# Autodesk Inventor assembly: Assembly1
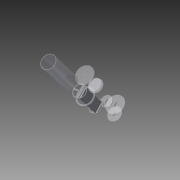
[picture p0: Inventor's stored thumbnail of the model, 180x180]
Saved by Autodesk Inventor 2015 (Build 190159000, 159)
## iProperties
Created: 2015-02-17
Part Number: Assembly1
Document SubType Name: Assembly
Designer: Hanjie
Author: Hanjie
## Documents named in this file (14)
- C:\Users\Qiuyang\Dropbox\VIP\SeaPerch\Dimensions\tube\Assembly1.iam
- C:\Users\Qiuyang\Dropbox\VIP\SeaPerch\Dimensions\tube\seal1.ipt
- C:\Users\Qiuyang\Dropbox\VIP\SeaPerch\Dimensions\tube\seal2.ipt
- C:\Users\Qiuyang\Dropbox\VIP\SeaPerch\Dimensions\tube\seal3.ipt
- C:\Users\Qiuyang\Dropbox\VIP\SeaPerch\Dimensions\tube\tube.ipt
- C:\Users\Qiuyang\Dropbox\VIP\SeaPerch\Dimensions\tube\open1.ipt
- C:\Users\Qiuyang\Dropbox\VIP\SeaPerch\Dimensions\tube\open2.ipt
- C:\Users\Qiuyang\Dropbox\VIP\SeaPerch\Dimensions\tube\open3.ipt
- C:\Users\Qiuyang\Dropbox\VIP\SeaPerch\Dimensions\tube\open4.ipt
- C:\Users\Qiuyang\Dropbox\VIP\SeaPerch\Dimensions\tube\open5.ipt
- C:\Users\Qiuyang\Dropbox\VIP\SeaPerch\Dimensions\tube\oringlarge.ipt
- C:\Users\Qiuyang\Dropbox\VIP\SeaPerch\Dimensions\tube\oringsmall.ipt
- C:\Users\Qiuyang\Dropbox\VIP\SeaPerch\Dimensions\tube\baseboard.ipt
- C:\Users\Qiuyang\Dropbox\VIP\SeaPerch\Dimensions\tube\fixpart.ipt
## Components (14 placed, 13 different names)
1. seal1:1 — Mate:2
2. seal2:1 — Mate:1, Mate:2
3. seal3:1 — Mate:1
4. tube:1
5. open1:1 — Angle:1, Angle:2
6. open2:1
7. open3:1
8. open4:1 — Angle:1, Angle:3
9. open5:1 — Angle:2
10. oringlarge:1 — Mate:11
11. oringsmall:1 — Mate:11
12. baseboard:1 — Mate:14, Mate:15
13. fixpart:1 — Mate:13, Mate:15
14. fixpart:2 — Mate:13, Mate:14, Angle:3
## Relationships (9: Mate 6, Angle 3)
- Mate:1: seal2:1 ↔ seal3:1
- Mate:2: seal1:1 ↔ seal2:1
- Mate:11: oringlarge:1 ↔ oringsmall:1
- Mate:13: fixpart:1 ↔ fixpart:2
- Mate:14: baseboard:1 ↔ fixpart:2
- Mate:15: baseboard:1 ↔ fixpart:1
- Angle:1 (0 deg): open1:1 ↔ open4:1
- Angle:2 (0 deg): open1:1 ↔ open5:1
- Angle:3 (0 deg): open4:1 ↔ fixpart:2
